# Autodesk Inventor assembly: HS 48T Gear, No Insert_mirrored
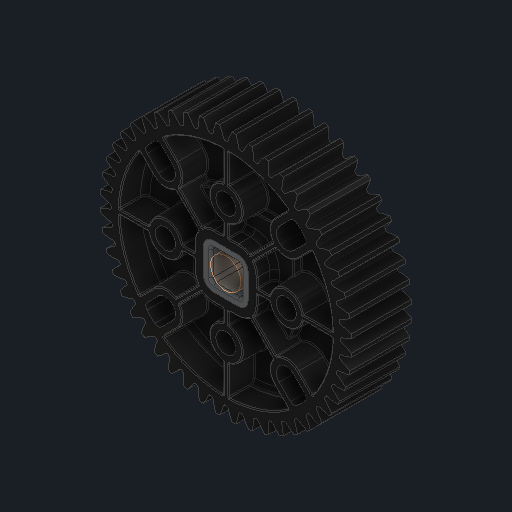
[picture p0: Inventor's stored thumbnail of the model, 512x512]
Saved by Autodesk Inventor 2024 (Build 280153000, 153)
## iProperties
Created: 2022-08-02
Part Number: HS 48T Gear, No Insert_mirrored
Document SubType Name: Assembly
Designer: Averey Ku
Author: ylu12
## Documents named in this file (2)
- D:\vex_robotics\hardware\cad\vroomba_v0.1\drivebay\mirrored_parts\HS 48T Gear, No Insert_mirrored.iam
- D:\vex_robotics\hardware\cad\vroomba_v0.1\drivebay\mirrored_parts\HS 48T Gear, No Insert_mirrored.ipt
## Components (1 placed, 1 different names)
1. HS 48T Gear, No Insert_mirrored:1 — Mate:12, Mate:11, Flush:6
## Relationships (3: Mate 2, Flush 1)
- Mate:12: HS 48T Gear, No Insert_mirrored:1
- Mate:11: HS 48T Gear, No Insert_mirrored:1
- Flush:6: HS 48T Gear, No Insert_mirrored:1
